# Autodesk Inventor assembly: Assembly1
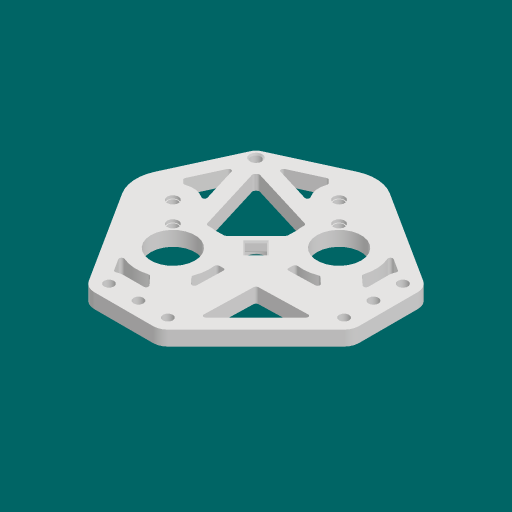
[picture p0: Inventor's stored thumbnail of the model, 512x512]
Saved by Autodesk Inventor 2023.1 (Build 271208000, 208)
## iProperties
Created: 2022-03-15
Part Number: Assembly1
Document SubType Name: Assembly
Designer: zac-h
Author: zac-h
## Documents named in this file (96)
- C:\Users\zac-h\Documents\CAD\guardSwerve1\Assembly1.iam
- C:\Users\zac-h\Documents\CAD\guardSwerve1\Undercarriage.ipt
- C:\Users\zac-h\Documents\CAD\VEX-CAD-Inventor-1.3.0\VEX-CAD-Inventor-1.3.0\Motion\Wheels\Tractions\2.75 Traction, No Insert.ipt
- C:\Users\zac-h\Documents\CAD\guardSwerve1\Assembly1\Design Accelerator\Bevel Gears1.iam
- C:\Users\zac-h\Documents\CAD\VEX-CAD-Inventor-1.3.0\VEX-CAD-Inventor-1.3.0\Motion\Pillow Bearing Block.ipt
- C:\Users\zac-h\Documents\CAD\VEX-CAD-Inventor-1.3.0\VEX-CAD-Inventor-1.3.0\Structure\Hardware\Screw Steel - Star\SScrew Star Smooth .750.ipt
- C:\Users\zac-h\Documents\CAD\VEX-CAD-Inventor-1.3.0\VEX-CAD-Inventor-1.3.0\Structure\Hardware\Screw Steel - Star.ipt
- C:\Users\zac-h\Documents\CAD\guardSwerve1\Assembly1\Design Accelerator\Bevel Gears1_MIR1.iam
- C:\Users\zac-h\Documents\CAD\VEX-CAD-Inventor-1.3.0\VEX-CAD-Inventor-1.3.0\Structure\Hardware\Nut Nylock.ipt
- C:\Users\zac-h\Documents\CAD\VEX-CAD-Inventor-1.3.0\VEX-CAD-Inventor-1.3.0\Electronics\V5 Simple Motor.ipt
- C:\Users\zac-h\Documents\CAD\guardSwerve1\608.ipt
- C:\Users\zac-h\Documents\CAD\guardSwerve1\bearingsleeve.ipt
- C:\Users\zac-h\Documents\CAD\guardSwerve1\lower_plate.ipt
- C:\Users\zac-h\Documents\CAD\guardSwerve1\Assembly1\Design Accelerator\Spur Gears1.iam
- C:\Users\zac-h\Documents\CAD\guardSwerve1\Assembly1\Design Accelerator\Spur Gears2.iam
- C:\Users\zac-h\Documents\CAD\guardSwerve1\Assembly1\Design Accelerator\Spur Gears3.iam
- C:\Users\zac-h\Documents\CAD\guardSwerve1\Assembly1\Design Accelerator\Spur Gears4.iam
- C:\Users\zac-h\Documents\CAD\VEX-CAD-Inventor-1.3.0\VEX-CAD-Inventor-1.3.0\Motion\Shaft LS\Shaft LS 2.5 in.ipt
- C:\Users\zac-h\Documents\CAD\VEX-CAD-Inventor-1.3.0\VEX-CAD-Inventor-1.3.0\Motion\Shaft LS.ipt
- C:\Users\zac-h\Documents\CAD\VEX-CAD-Inventor-1.3.0\VEX-CAD-Inventor-1.3.0\Motion\Shaft Collar with Set Screw.ipt
- C:\Users\zac-h\Documents\CAD\guardSwerve1\vroller.ipt
- C:\Users\zac-h\Documents\CAD\guardSwerve1\upper.ipt
- C:\Users\zac-h\Documents\CAD\guardSwerve1\uppermidblock.ipt
- C:\Users\zac-h\Documents\CAD\guardSwerve1\motorplate.ipt
- C:\Users\zac-h\Documents\CAD\guardSwerve1\Assembly2.iam
- C:\Users\zac-h\Documents\CAD\guardSwerve1\Assembly3.iam
- C:\Users\zac-h\Documents\CAD\guardSwerve1\stls\encoderring.ipt
- C:\Users\zac-h\Documents\CAD\VEX-CAD-Inventor-1.3.0\VEX-CAD-Inventor-1.3.0\Structure\C-Channels\Aluminum 1x2x1\Alu C 1x2x1x26.ipt
- C:\Users\zac-h\Documents\CAD\guardSwerve1\Undercarriage_MIR.ipt
- C:\Users\zac-h\Documents\CAD\VEX-CAD-Inventor-1.3.0\VEX-CAD-Inventor-1.3.0\Motion\Wheels\Tractions\2.75 Traction, No Insert_MIR.ipt
- C:\Users\zac-h\Documents\CAD\guardSwerve1\Assembly1\Design Accelerator\Bevel Gears1_MIR2.iam
- C:\Users\zac-h\Documents\CAD\VEX-CAD-Inventor-1.3.0\VEX-CAD-Inventor-1.3.0\Motion\Pillow Bearing Block_MIR.ipt
- C:\Users\zac-h\Documents\CAD\guardSwerve1\Assembly1\Design Accelerator\Bevel Gears1_MIR1_MIR.iam
- C:\Users\zac-h\Documents\CAD\VEX-CAD-Inventor-1.3.0\VEX-CAD-Inventor-1.3.0\Structure\Hardware\Nut Nylock_MIR.ipt
- C:\Users\zac-h\Documents\CAD\VEX-CAD-Inventor-1.3.0\VEX-CAD-Inventor-1.3.0\Electronics\V5 Simple Motor_MIR.ipt
- C:\Users\zac-h\Documents\CAD\guardSwerve1\608_MIR.ipt
- C:\Users\zac-h\Documents\CAD\guardSwerve1\bearingsleeve_MIR.ipt
- C:\Users\zac-h\Documents\CAD\guardSwerve1\lower_plate_MIR.ipt
- C:\Users\zac-h\Documents\CAD\guardSwerve1\Assembly1\Design Accelerator\Spur Gears1_MIR.iam
- C:\Users\zac-h\Documents\CAD\guardSwerve1\Assembly1\Design Accelerator\Spur Gears2_MIR.iam
- C:\Users\zac-h\Documents\CAD\guardSwerve1\Assembly1\Design Accelerator\Spur Gears3_MIR.iam
- C:\Users\zac-h\Documents\CAD\guardSwerve1\Assembly1\Design Accelerator\Spur Gears4_MIR.iam
- C:\Users\zac-h\Documents\CAD\VEX-CAD-Inventor-1.3.0\VEX-CAD-Inventor-1.3.0\Motion\Shaft Collar with Set Screw_MIR.ipt
- C:\Users\zac-h\Documents\CAD\guardSwerve1\vroller_MIR.ipt
- C:\Users\zac-h\Documents\CAD\guardSwerve1\upper_MIR.ipt
- C:\Users\zac-h\Documents\CAD\guardSwerve1\uppermidblock_MIR.ipt
- C:\Users\zac-h\Documents\CAD\guardSwerve1\motorplate_MIR.ipt
- C:\Users\zac-h\Documents\CAD\guardSwerve1\Assembly2_MIR.iam
- C:\Users\zac-h\Documents\CAD\guardSwerve1\Assembly3_MIR.iam
- C:\Users\zac-h\Documents\CAD\guardSwerve1\stls\encoderring_MIR.ipt
- C:\Users\zac-h\Documents\CAD\guardSwerve1\Undercarriage_MIR1.ipt
- C:\Users\zac-h\Documents\CAD\VEX-CAD-Inventor-1.3.0\VEX-CAD-Inventor-1.3.0\Motion\Wheels\Tractions\2.75 Traction, No Insert_MIR1.ipt
- C:\Users\zac-h\Documents\CAD\guardSwerve1\Assembly1\Design Accelerator\Bevel Gears1_MIR3.iam
- C:\Users\zac-h\Documents\CAD\VEX-CAD-Inventor-1.3.0\VEX-CAD-Inventor-1.3.0\Motion\Pillow Bearing Block_MIR1.ipt
- C:\Users\zac-h\Documents\CAD\guardSwerve1\Assembly1\Design Accelerator\Bevel Gears1_MIR1_MIR1.iam
- C:\Users\zac-h\Documents\CAD\VEX-CAD-Inventor-1.3.0\VEX-CAD-Inventor-1.3.0\Structure\Hardware\Nut Nylock_MIR1.ipt
- C:\Users\zac-h\Documents\CAD\VEX-CAD-Inventor-1.3.0\VEX-CAD-Inventor-1.3.0\Electronics\V5 Simple Motor_MIR1.ipt
- C:\Users\zac-h\Documents\CAD\guardSwerve1\608_MIR1.ipt
- C:\Users\zac-h\Documents\CAD\guardSwerve1\bearingsleeve_MIR1.ipt
- C:\Users\zac-h\Documents\CAD\guardSwerve1\lower_plate_MIR1.ipt
- C:\Users\zac-h\Documents\CAD\guardSwerve1\Assembly1\Design Accelerator\Spur Gears1_MIR1.iam
- C:\Users\zac-h\Documents\CAD\guardSwerve1\Assembly1\Design Accelerator\Spur Gears2_MIR1.iam
- C:\Users\zac-h\Documents\CAD\guardSwerve1\Assembly1\Design Accelerator\Spur Gears3_MIR1.iam
- C:\Users\zac-h\Documents\CAD\guardSwerve1\Assembly1\Design Accelerator\Spur Gears4_MIR1.iam
- C:\Users\zac-h\Documents\CAD\VEX-CAD-Inventor-1.3.0\VEX-CAD-Inventor-1.3.0\Motion\Shaft Collar with Set Screw_MIR1.ipt
- C:\Users\zac-h\Documents\CAD\guardSwerve1\vroller_MIR1.ipt
- C:\Users\zac-h\Documents\CAD\guardSwerve1\upper_MIR1.ipt
- C:\Users\zac-h\Documents\CAD\guardSwerve1\uppermidblock_MIR1.ipt
- C:\Users\zac-h\Documents\CAD\guardSwerve1\motorplate_MIR1.ipt
- C:\Users\zac-h\Documents\CAD\guardSwerve1\Assembly2_MIR1.iam
- C:\Users\zac-h\Documents\CAD\guardSwerve1\Assembly3_MIR1.iam
- C:\Users\zac-h\Documents\CAD\guardSwerve1\stls\encoderring_MIR1.ipt
- C:\Users\zac-h\Documents\CAD\VEX-CAD-Inventor-1.3.0\VEX-CAD-Inventor-1.3.0\Structure\C-Channels\Aluminum 1x2x1\Alu C 1x2x1x26_MIR.ipt
- C:\Users\zac-h\Documents\CAD\guardSwerve1\Undercarriage_MIR_MIR.ipt
- C:\Users\zac-h\Documents\CAD\VEX-CAD-Inventor-1.3.0\VEX-CAD-Inventor-1.3.0\Motion\Wheels\Tractions\2.75 Traction, No Insert_MIR_MIR.ipt
- C:\Users\zac-h\Documents\CAD\guardSwerve1\Assembly1\Design Accelerator\Bevel Gears1_MIR2_MIR.iam
- C:\Users\zac-h\Documents\CAD\VEX-CAD-Inventor-1.3.0\VEX-CAD-Inventor-1.3.0\Motion\Pillow Bearing Block_MIR_MIR.ipt
- C:\Users\zac-h\Documents\CAD\guardSwerve1\Assembly1\Design Accelerator\Bevel Gears1_MIR1_MIR_MIR.iam
- C:\Users\zac-h\Documents\CAD\VEX-CAD-Inventor-1.3.0\VEX-CAD-Inventor-1.3.0\Structure\Hardware\Nut Nylock_MIR_MIR.ipt
- C:\Users\zac-h\Documents\CAD\VEX-CAD-Inventor-1.3.0\VEX-CAD-Inventor-1.3.0\Electronics\V5 Simple Motor_MIR_MIR.ipt
- C:\Users\zac-h\Documents\CAD\guardSwerve1\608_MIR_MIR.ipt
- C:\Users\zac-h\Documents\CAD\guardSwerve1\bearingsleeve_MIR_MIR.ipt
- C:\Users\zac-h\Documents\CAD\guardSwerve1\lower_plate_MIR_MIR.ipt
- C:\Users\zac-h\Documents\CAD\guardSwerve1\Assembly1\Design Accelerator\Spur Gears1_MIR_MIR.iam
- C:\Users\zac-h\Documents\CAD\guardSwerve1\Assembly1\Design Accelerator\Spur Gears2_MIR_MIR.iam
- C:\Users\zac-h\Documents\CAD\guardSwerve1\Assembly1\Design Accelerator\Spur Gears3_MIR_MIR.iam
- C:\Users\zac-h\Documents\CAD\guardSwerve1\Assembly1\Design Accelerator\Spur Gears4_MIR_MIR.iam
- C:\Users\zac-h\Documents\CAD\VEX-CAD-Inventor-1.3.0\VEX-CAD-Inventor-1.3.0\Motion\Shaft Collar with Set Screw_MIR_MIR.ipt
- C:\Users\zac-h\Documents\CAD\guardSwerve1\upper_MIR_MIR.ipt
- C:\Users\zac-h\Documents\CAD\guardSwerve1\uppermidblock_MIR_MIR.ipt
- C:\Users\zac-h\Documents\CAD\guardSwerve1\motorplate_MIR_MIR.ipt
- C:\Users\zac-h\Documents\CAD\guardSwerve1\Assembly2_MIR_MIR.iam
- C:\Users\zac-h\Documents\CAD\guardSwerve1\Assembly3_MIR_MIR.iam
- C:\Users\zac-h\Documents\CAD\guardSwerve1\stls\encoderring_MIR_MIR.ipt
- C:\Users\zac-h\Documents\CAD\guardSwerve1\vroller_MIR_MIR.ipt
- C:\Users\zac-h\Documents\CAD\VEX-CAD-Inventor-1.3.0\VEX-CAD-Inventor-1.3.0\Structure\C-Channels\Aluminum 1x2x1\Alu C 1x2x1x26_MIR_MIR.ipt
## Components (189 placed, 90 different names)
1. Undercarriage:1 — Mate:1, Insert:1, Insert:2, Insert:3, Insert:4, Insert:5, Insert:6, Insert:7, Insert:8, Flush:1, Insert:13, Insert:14, Flush:2, Flush:3, Insert:19, Mate:42, Mate:46, Mate:50, Mate:53, Flush:11
2. 2.75 Traction, No Insert:1 — Rigid:1, Mate:1, Mate:4
3. Bevel Gears:1 [sub-assembly] — Rigid:1, Mate:2, Mate:3, Angle:1, Angle:2
4. Pillow Bearing Block:1 — Insert:5, Insert:6, Insert:9, Insert:10, Insert:28
5. Pillow Bearing Block:2 — Insert:1, Insert:2, Mate:2, Insert:11, Insert:12, Insert:29
6. SScrew Star Smooth .750:1 — Insert:3
7. SScrew Star Smooth .750:2 — Insert:4
8. SScrew Star Smooth .750:3 — Insert:7
9. SScrew Star Smooth .750:4 — Insert:8
10. Bevel Gears1_MIR1:1 [sub-assembly] — Mate:3, Angle:1, Mate:4
11. Nut Nylock:1 — Insert:9
12. Nut Nylock:2 — Insert:11
13. Nut Nylock:3 — Insert:10
14. Nut Nylock:4 — Insert:12
15. V5 Simple Motor:1 — Insert:39, Insert:40
16. V5 Simple Motor:2 — Insert:37, Insert:38
17. 608:1 — Flush:1, Insert:14, Insert:21
18. 608:2 — Insert:13, Insert:15
19. bearingsleeve:1 — Insert:15, Mate:44, Mate:47
20. lower_plate:1 — Flush:2, Flush:3, Insert:32, Insert:33, Insert:34, Flush:6, Flush:7, Insert:41, Insert:42, Insert:43
21. Spur Gears:1 [sub-assembly] — Mate:44, Mate:45, Mate:46, Mate:47, Mate:49, Mate:51
22. 608:3 — Insert:19, Insert:20
23. bearingsleeve:2 — Insert:20, Mate:45
24. bearingsleeve:3 — Insert:21, Mate:48
25. Spur Gears:2 [sub-assembly] — Mate:48, Mate:49, Mate:50, Mate:51, Insert:31, Mate:54
26. Spur Gears:3 [sub-assembly] — Insert:26, Mate:53, Mate:54
27. 608:4 — Insert:24, Insert:31
28. 608:5 — Insert:25, Insert:26
29. bearingsleeve:4 — Insert:24
30. bearingsleeve:5 — Insert:25, Mate:43
31. Spur Gears:4 [sub-assembly] — Mate:42, Mate:43, Mate:52
32. Shaft LS 2.5 in:1 — Insert:30
33. Shaft Collar with Set Screw:1 — Insert:29, Insert:30
34. Shaft Collar with Set Screw:2 — Insert:28
35. 608:6 — Insert:32
36. 608:7 — Insert:33
37. 608:8 — Insert:34, Flush:4, Flush:5, Insert:36
38. midblock — Flush:6, Flush:7, Flush:8, Flush:9
39. uppermidblock:1 — Flush:8, Flush:9, Flush:10, Angle:3
40. motorplate:1 — Flush:10, Insert:37, Insert:38, Insert:39, Insert:40
41. Assembly2:1 [sub-assembly]
42. Assembly3:1 [sub-assembly]
43. encoderring:1 — Flush:11
44. Alu C 1x2x1x26:1 — Insert:41
45. Alu C 1x2x1x26:2 — Insert:42, Insert:43
46. Undercarriage_MIR:1 — Mate:55, Insert:44, Insert:45, Insert:46, Insert:47, Insert:48, Insert:49, Insert:50, Insert:51, Insert:56, Mate:59, Insert:57, Mate:60, Mate:61, Mate:63, Insert:59, Mate:67, Mate:71, Mate:73, Mate:82
47. 2.75 Traction, No Insert_MIR:1 — Mate:55, Mate:57, Rigid:2
48. Bevel Gears1_MIR2:1 [sub-assembly] — Mate:56, Mate:58, Angle:4, Angle:5, Rigid:2
49. Pillow Bearing Block_MIR:1 — Insert:44, Insert:45, Insert:52, Insert:54, Insert:68
50. Pillow Bearing Block_MIR:2 — Mate:56, Insert:46, Insert:47, Insert:53, Insert:55, Insert:67
51. SScrew Star Smooth .750:5 — Insert:48
52. SScrew Star Smooth .750:6 — Insert:49
53. SScrew Star Smooth .750:7 — Insert:50
54. SScrew Star Smooth .750:8 — Insert:51
55. Bevel Gears1_MIR1_MIR:1 [sub-assembly] — Mate:57, Mate:58, Angle:4
56. Nut Nylock_MIR:1 — Insert:52
57. Nut Nylock_MIR:2 — Insert:53
58. Nut Nylock_MIR:3 — Insert:54
59. Nut Nylock_MIR:4 — Insert:55
60. V5 Simple Motor_MIR:1 — Insert:73, Insert:74
61. V5 Simple Motor_MIR:2 — Insert:75, Insert:76
62. 608_MIR:1 — Insert:56, Mate:59, Insert:61
63. 608_MIR:2 — Insert:57, Insert:58
64. bearingsleeve_MIR:1 — Insert:58, Mate:62, Mate:64
65. lower_plate_MIR:1 — Mate:60, Mate:61, Insert:69, Insert:70, Insert:71, Mate:76, Mate:77
66. Spur Gears1_MIR:1 [sub-assembly] — Mate:62, Mate:63, Mate:64, Mate:65, Mate:66, Mate:68
67. 608_MIR:3 — Insert:59, Insert:60
68. bearingsleeve_MIR:2 — Mate:65, Insert:60
69. bearingsleeve_MIR:3 — Insert:61, Mate:69
70. Spur Gears2_MIR:1 [sub-assembly] — Mate:66, Mate:67, Mate:68, Mate:69, Mate:70, Insert:62
71. Spur Gears3_MIR:1 [sub-assembly] — Mate:70, Mate:71, Insert:63
72. 608_MIR:4 — Insert:62, Insert:64
73. 608_MIR:5 — Insert:63, Insert:65
74. bearingsleeve_MIR:4 — Insert:64
75. bearingsleeve_MIR:5 — Insert:65, Mate:72
76. Spur Gears4_MIR:1 [sub-assembly] — Mate:72, Mate:73, Mate:81
77. Shaft LS 2.5 in:2 — Insert:66
78. Shaft Collar with Set Screw_MIR:1 — Insert:66, Insert:67
79. Shaft Collar with Set Screw_MIR:2 — Insert:68
80. 608_MIR:6 — Insert:69
81. 608_MIR:7 — Insert:70
82. 608_MIR:8 — Insert:71, Insert:72, Mate:74, Mate:75
83. upper_MIR:1 — Mate:76, Mate:77, Mate:78, Mate:79
84. uppermidblock_MIR:1 — Mate:78, Mate:79, Mate:80, Angle:6
85. motorplate_MIR:1 — Insert:73, Insert:74, Insert:75, Insert:76, Mate:80
86. Assembly2_MIR:1 [sub-assembly]
87. Assembly3_MIR:1 [sub-assembly]
88. encoderring_MIR:1 — Mate:82
89. Undercarriage_MIR1:1 — Mate:83, Insert:77, Insert:78, Insert:79, Insert:80, Insert:81, Insert:82, Insert:83, Insert:84, Insert:89, Mate:87, Insert:90, Mate:88, Mate:89, Mate:91, Insert:92, Mate:95, Mate:99, Mate:101, Mate:110
90. 2.75 Traction, No Insert_MIR1:1 — Mate:83, Mate:85, Rigid:3
91. Bevel Gears1_MIR3:1 [sub-assembly] — Mate:84, Mate:86, Angle:7, Angle:8, Rigid:3
92. Pillow Bearing Block_MIR1:1 — Insert:77, Insert:78, Insert:85, Insert:87, Insert:101
93. Pillow Bearing Block_MIR1:2 — Mate:84, Insert:79, Insert:80, Insert:86, Insert:88, Insert:100
94. SScrew Star Smooth .750:9 — Insert:81
95. SScrew Star Smooth .750:10 — Insert:82
96. SScrew Star Smooth .750:11 — Insert:83
97. SScrew Star Smooth .750:12 — Insert:84
98. Bevel Gears1_MIR1_MIR1:1 [sub-assembly] — Mate:85, Mate:86, Angle:7
99. Nut Nylock_MIR1:1 — Insert:85
100. Nut Nylock_MIR1:2 — Insert:86
101. Nut Nylock_MIR1:3 — Insert:87
102. Nut Nylock_MIR1:4 — Insert:88
103. V5 Simple Motor_MIR1:1 — Insert:106, Insert:107
104. V5 Simple Motor_MIR1:2 — Insert:108, Insert:109
105. 608_MIR1:1 — Insert:89, Mate:87, Insert:94
106. 608_MIR1:2 — Insert:90, Insert:91
107. bearingsleeve_MIR1:1 — Insert:91, Mate:90, Mate:92
108. lower_plate_MIR1:1 — Mate:88, Mate:89, Insert:102, Insert:103, Insert:104, Mate:104, Mate:105, Insert:110, Insert:111, Insert:112
109. Spur Gears1_MIR1:1 [sub-assembly] — Mate:90, Mate:91, Mate:92, Mate:93, Mate:94, Mate:96
110. 608_MIR1:3 — Insert:92, Insert:93
111. bearingsleeve_MIR1:2 — Mate:93, Insert:93
112. bearingsleeve_MIR1:3 — Insert:94, Mate:97
113. Spur Gears2_MIR1:1 [sub-assembly] — Mate:94, Mate:95, Mate:96, Mate:97, Mate:98, Insert:95
114. Spur Gears3_MIR1:1 [sub-assembly] — Mate:98, Mate:99, Insert:96
115. 608_MIR1:4 — Insert:95, Insert:97
116. 608_MIR1:5 — Insert:96, Insert:98
117. bearingsleeve_MIR1:4 — Insert:97
118. bearingsleeve_MIR1:5 — Insert:98, Mate:100
119. Spur Gears4_MIR1:1 [sub-assembly] — Mate:100, Mate:101, Mate:109
120. Shaft LS 2.5 in:3 — Insert:99
121. Shaft Collar with Set Screw_MIR1:1 — Insert:99, Insert:100
122. Shaft Collar with Set Screw_MIR1:2 — Insert:101
123. 608_MIR1:6 — Insert:102
124. 608_MIR1:7 — Insert:103
125. 608_MIR1:8 — Insert:104, Insert:105, Mate:102, Mate:103
126. upper_MIR1:1 — Mate:104, Mate:105, Mate:106, Mate:107
127. uppermidblock_MIR1:1 — Mate:106, Mate:107, Mate:108, Angle:9
128. motorplate_MIR1:1 — Insert:106, Insert:107, Insert:108, Insert:109, Mate:108
129. Assembly2_MIR1:1 [sub-assembly]
130. Assembly3_MIR1:1 [sub-assembly]
131. encoderring_MIR1:1 — Mate:110
132. Alu C 1x2x1x26_MIR:1 — Insert:110
133. Alu C 1x2x1x26_MIR:2 — Insert:111, Insert:112
134. Undercarriage_MIR_MIR:1 — Mate:111, Insert:113, Insert:114, Insert:115, Insert:116, Insert:117, Insert:118, Insert:119, Insert:120, Flush:12, Insert:125, Insert:126, Flush:13, Flush:14, Mate:116, Insert:128, Mate:121, Mate:123, Mate:125, Flush:22
135. 2.75 Traction, No Insert_MIR_MIR:1 — Mate:111, Mate:114, Rigid:4
136. Bevel Gears1_MIR2_MIR:1 [sub-assembly] — Mate:112, Mate:113, Angle:10, Angle:11, Rigid:4
137. Pillow Bearing Block_MIR_MIR:1 — Insert:113, Insert:114, Insert:121, Insert:123, Insert:137
138. Pillow Bearing Block_MIR_MIR:2 — Insert:115, Insert:116, Mate:112, Insert:122, Insert:124, Insert:135
139. SScrew Star Smooth .750:13 — Insert:117
140. SScrew Star Smooth .750:14 — Insert:118
141. SScrew Star Smooth .750:15 — Insert:119
142. SScrew Star Smooth .750:16 — Insert:120
143. Bevel Gears1_MIR1_MIR_MIR:1 [sub-assembly] — Mate:113, Mate:114, Angle:10
144. Nut Nylock_MIR_MIR:1 — Insert:121
145. Nut Nylock_MIR_MIR:2 — Insert:122
146. Nut Nylock_MIR_MIR:3 — Insert:123
147. Nut Nylock_MIR_MIR:4 — Insert:124
148. V5 Simple Motor_MIR_MIR:1 — Insert:144, Insert:145
149. V5 Simple Motor_MIR_MIR:2 — Insert:142, Insert:143
150. 608_MIR_MIR:1 — Flush:12, Insert:125, Insert:130
151. 608_MIR_MIR:2 — Insert:126, Insert:127
152. bearingsleeve_MIR_MIR:1 — Insert:127, Mate:115, Mate:117
153. lower_plate_MIR_MIR:1 — Flush:13, Flush:14, Insert:138, Insert:139, Insert:140, Flush:17, Flush:18
154. Spur Gears1_MIR_MIR:1 [sub-assembly] — Mate:115, Mate:116, Mate:117, Mate:118, Mate:120, Mate:122
155. 608_MIR_MIR:3 — Insert:128, Insert:129
156. bearingsleeve_MIR_MIR:2 — Insert:129, Mate:118
157. bearingsleeve_MIR_MIR:3 — Insert:130, Mate:119
158. Spur Gears2_MIR_MIR:1 [sub-assembly] — Mate:119, Mate:120, Mate:121, Mate:122, Mate:124, Insert:131
159. Spur Gears3_MIR_MIR:1 [sub-assembly] — Mate:123, Mate:124, Insert:132
160. 608_MIR_MIR:4 — Insert:131, Insert:133
161. 608_MIR_MIR:5 — Insert:132, Insert:134
162. bearingsleeve_MIR_MIR:4 — Insert:133
163. bearingsleeve_MIR_MIR:5 — Insert:134, Mate:126
164. Spur Gears4_MIR_MIR:1 [sub-assembly] — Mate:125, Mate:126, Mate:127
165. Shaft LS 2.5 in:4 — Insert:136
166. Shaft Collar with Set Screw_MIR_MIR:1 — Insert:135, Insert:136
167. Shaft Collar with Set Screw_MIR_MIR:2 — Insert:137
168. 608_MIR_MIR:6 — Insert:138
169. 608_MIR_MIR:7 — Insert:139
170. 608_MIR_MIR:8 — Insert:140, Flush:15, Flush:16, Insert:141
171. upper_MIR_MIR:1 — Flush:17, Flush:18, Flush:19, Flush:20
172. uppermidblock_MIR_MIR:1 — Flush:19, Flush:20, Flush:21, Angle:12
173. motorplate_MIR_MIR:1 — Flush:21, Insert:142, Insert:143, Insert:144, Insert:145
174. Assembly2_MIR_MIR:1 [sub-assembly]
175. Assembly3_MIR_MIR:1 [sub-assembly]
176. encoderring_MIR_MIR:1 — Flush:22
177. Alu C 1x2x1x26_MIR_MIR:1
178. vroller:1 — Flush:4, Flush:5, Insert:36
179. vroller:2
180. vroller:3
181. vroller_MIR:1 — Insert:72, Mate:74, Mate:75
182. vroller_MIR:2
183. vroller_MIR:3
184. vroller_MIR1:1 — Insert:105, Mate:102, Mate:103
185. vroller_MIR1:2
186. vroller_MIR1:3
187. vroller_MIR_MIR:1 — Flush:15, Flush:16, Insert:141
188. vroller_MIR_MIR:2
189. vroller_MIR_MIR:3
## Component patterns: (3 elements, first: vroller:1), (3 elements, first: vroller_MIR:1), (3 elements, first: vroller_MIR1:1), (3 elements, first: vroller_MIR_MIR:1)
## Relationships (266: Insert 138, Mate 90, Flush 22, Angle 12, WeldJoint 4)
- Rigid:1 [WeldJoint]: 2.75 Traction, No Insert:1 ↔ Bevel Gears:1
- Mate:1: Undercarriage:1 ↔ 2.75 Traction, No Insert:1
- Insert:1: Undercarriage:1 ↔ Pillow Bearing Block:2
- Insert:2: Undercarriage:1 ↔ Pillow Bearing Block:2
- Mate:2: Bevel Gears:1 ↔ Pillow Bearing Block:2
- Insert:3: Undercarriage:1 ↔ SScrew Star Smooth .750:1
- Insert:4: Undercarriage:1 ↔ SScrew Star Smooth .750:2
- Mate:3: Bevel Gears:1 ↔ Bevel Gears1_MIR1:1
- Angle:1 (0 deg): Bevel Gears:1 ↔ Bevel Gears1_MIR1:1
- Mate:4: 2.75 Traction, No Insert:1 ↔ Bevel Gears1_MIR1:1
- Angle:2 (180 deg): Bevel Gears:1
- Insert:5: Undercarriage:1 ↔ Pillow Bearing Block:1
- Insert:6: Undercarriage:1 ↔ Pillow Bearing Block:1
- Insert:7: Undercarriage:1 ↔ SScrew Star Smooth .750:3
- Insert:8: Undercarriage:1 ↔ SScrew Star Smooth .750:4
- Insert:9: Pillow Bearing Block:1 ↔ Nut Nylock:1
- Insert:10: Pillow Bearing Block:1 ↔ Nut Nylock:3
- Insert:11: Pillow Bearing Block:2 ↔ Nut Nylock:2
- Insert:12: Pillow Bearing Block:2 ↔ Nut Nylock:4
- Flush:1: Undercarriage:1 ↔ 608:1
- Insert:13: Undercarriage:1 ↔ 608:2
- Insert:14: Undercarriage:1 ↔ 608:1
- Insert:15: 608:2 ↔ bearingsleeve:1
- Flush:2: Undercarriage:1 ↔ lower_plate:1
- Flush:3 (3 mm): Undercarriage:1 ↔ lower_plate:1
- Insert:19: Undercarriage:1 ↔ 608:3
- Insert:20: 608:3 ↔ bearingsleeve:2
- Insert:21: 608:1 ↔ bearingsleeve:3
- Insert:24: 608:4 ↔ bearingsleeve:4
- Insert:25: 608:5 ↔ bearingsleeve:5
- Mate:42: Undercarriage:1 ↔ Spur Gears:4
- Mate:43: bearingsleeve:5 ↔ Spur Gears:4
- Insert:26: Spur Gears:3 ↔ 608:5
- Insert:28: Pillow Bearing Block:1 ↔ Shaft Collar with Set Screw:2
- Insert:29: Pillow Bearing Block:2 ↔ Shaft Collar with Set Screw:1
- Insert:30: Shaft LS 2.5 in:1 ↔ Shaft Collar with Set Screw:1
- Mate:44: bearingsleeve:1 ↔ Spur Gears:1
- Mate:45 (1.5875 mm): Spur Gears:1 ↔ bearingsleeve:2
- Mate:46: Undercarriage:1 ↔ Spur Gears:1
- Mate:47 (1.5875 mm): bearingsleeve:1 ↔ Spur Gears:1
- Mate:48: bearingsleeve:3 ↔ Spur Gears:2
- Mate:49 (1.5875 mm): Spur Gears:1 ↔ Spur Gears:2
- Mate:50: Undercarriage:1 ↔ Spur Gears:2
- Mate:51 (1.5875 mm): Spur Gears:1 ↔ Spur Gears:2
- Insert:31: Spur Gears:2 ↔ 608:4
- Insert:32: lower_plate:1 ↔ 608:6
- Insert:33: lower_plate:1 ↔ 608:7
- Insert:34: lower_plate:1 ↔ 608:8
- Flush:4: 608:8 ↔ vroller:1
- Flush:5: 608:8 ↔ vroller:1
- Flush:6: lower_plate:1 ↔ midblock
- Flush:7: lower_plate:1 ↔ midblock
- Insert:36: 608:8 ↔ vroller:1
- Flush:8: midblock ↔ uppermidblock:1
- Flush:9: midblock ↔ uppermidblock:1
- Flush:10: uppermidblock:1 ↔ motorplate:1
- Insert:37: V5 Simple Motor:2 ↔ motorplate:1
- Insert:38: V5 Simple Motor:2 ↔ motorplate:1
- Insert:39: V5 Simple Motor:1 ↔ motorplate:1
- Insert:40: V5 Simple Motor:1 ↔ motorplate:1
- Mate:52: Spur Gears:4
- Angle:3 (90 deg): uppermidblock:1
- Mate:53: Undercarriage:1 ↔ Spur Gears:3
- Mate:54: Spur Gears:2 ↔ Spur Gears:3
- Flush:11: Undercarriage:1 ↔ encoderring:1
- Insert:41: lower_plate:1 ↔ Alu C 1x2x1x26:1
- Insert:42: lower_plate:1 ↔ Alu C 1x2x1x26:2
- Insert:43: lower_plate:1 ↔ Alu C 1x2x1x26:2
- Mate:55: Undercarriage_MIR:1 ↔ 2.75 Traction, No Insert_MIR:1
- Insert:44: Undercarriage_MIR:1 ↔ Pillow Bearing Block_MIR:1
- Insert:45: Undercarriage_MIR:1 ↔ Pillow Bearing Block_MIR:1
- Mate:56: Bevel Gears1_MIR2:1 ↔ Pillow Bearing Block_MIR:2
- Insert:46: Undercarriage_MIR:1 ↔ Pillow Bearing Block_MIR:2
- Insert:47: Undercarriage_MIR:1 ↔ Pillow Bearing Block_MIR:2
- Insert:48: Undercarriage_MIR:1 ↔ SScrew Star Smooth .750:5
- Insert:49: Undercarriage_MIR:1 ↔ SScrew Star Smooth .750:6
- Insert:50: Undercarriage_MIR:1 ↔ SScrew Star Smooth .750:7
- Insert:51: Undercarriage_MIR:1 ↔ SScrew Star Smooth .750:8
- Mate:57: 2.75 Traction, No Insert_MIR:1 ↔ Bevel Gears1_MIR1_MIR:1
- Mate:58: Bevel Gears1_MIR2:1 ↔ Bevel Gears1_MIR1_MIR:1
- Angle:4 (0 deg): Bevel Gears1_MIR2:1 ↔ Bevel Gears1_MIR1_MIR:1
- Angle:5 (180 deg): Bevel Gears1_MIR2:1
- Insert:52: Pillow Bearing Block_MIR:1 ↔ Nut Nylock_MIR:1
- Insert:53: Pillow Bearing Block_MIR:2 ↔ Nut Nylock_MIR:2
- Insert:54: Pillow Bearing Block_MIR:1 ↔ Nut Nylock_MIR:3
- Insert:55: Pillow Bearing Block_MIR:2 ↔ Nut Nylock_MIR:4
- Insert:56: Undercarriage_MIR:1 ↔ 608_MIR:1
- Mate:59: Undercarriage_MIR:1 ↔ 608_MIR:1
- Insert:57: Undercarriage_MIR:1 ↔ 608_MIR:2
- Insert:58: 608_MIR:2 ↔ bearingsleeve_MIR:1
- Mate:60 (3 mm): Undercarriage_MIR:1 ↔ lower_plate_MIR:1
- Mate:61: Undercarriage_MIR:1 ↔ lower_plate_MIR:1
- Mate:62 (1.5875 mm): bearingsleeve_MIR:1 ↔ Spur Gears1_MIR:1
- Mate:63: Undercarriage_MIR:1 ↔ Spur Gears1_MIR:1
- Mate:64: bearingsleeve_MIR:1 ↔ Spur Gears1_MIR:1
- Insert:59: Undercarriage_MIR:1 ↔ 608_MIR:3
- Mate:65 (1.5875 mm): Spur Gears1_MIR:1 ↔ bearingsleeve_MIR:2
- Insert:60: 608_MIR:3 ↔ bearingsleeve_MIR:2
- Insert:61: 608_MIR:1 ↔ bearingsleeve_MIR:3
- Mate:66 (1.5875 mm): Spur Gears1_MIR:1 ↔ Spur Gears2_MIR:1
- Mate:67: Undercarriage_MIR:1 ↔ Spur Gears2_MIR:1
- Mate:68 (1.5875 mm): Spur Gears1_MIR:1 ↔ Spur Gears2_MIR:1
- Mate:69: bearingsleeve_MIR:3 ↔ Spur Gears2_MIR:1
- Mate:70: Spur Gears2_MIR:1 ↔ Spur Gears3_MIR:1
- Mate:71: Undercarriage_MIR:1 ↔ Spur Gears3_MIR:1
- Insert:62: Spur Gears2_MIR:1 ↔ 608_MIR:4
- Insert:63: Spur Gears3_MIR:1 ↔ 608_MIR:5
- Insert:64: 608_MIR:4 ↔ bearingsleeve_MIR:4
- Insert:65: 608_MIR:5 ↔ bearingsleeve_MIR:5
- Mate:72: bearingsleeve_MIR:5 ↔ Spur Gears4_MIR:1
- Mate:73: Undercarriage_MIR:1 ↔ Spur Gears4_MIR:1
- Insert:66: Shaft LS 2.5 in:2 ↔ Shaft Collar with Set Screw_MIR:1
- Insert:67: Pillow Bearing Block_MIR:2 ↔ Shaft Collar with Set Screw_MIR:1
- Insert:68: Pillow Bearing Block_MIR:1 ↔ Shaft Collar with Set Screw_MIR:2
- Insert:69: lower_plate_MIR:1 ↔ 608_MIR:6
- Insert:70: lower_plate_MIR:1 ↔ 608_MIR:7
- Insert:71: lower_plate_MIR:1 ↔ 608_MIR:8
- Insert:72: 608_MIR:8 ↔ vroller_MIR:1
- Mate:74: 608_MIR:8 ↔ vroller_MIR:1
- Mate:75: 608_MIR:8 ↔ vroller_MIR:1
- Mate:76: lower_plate_MIR:1 ↔ upper_MIR:1
- Mate:77: lower_plate_MIR:1 ↔ upper_MIR:1
- Mate:78: upper_MIR:1 ↔ uppermidblock_MIR:1
- Mate:79: upper_MIR:1 ↔ uppermidblock_MIR:1
- Insert:73: V5 Simple Motor_MIR:1 ↔ motorplate_MIR:1
- Insert:74: V5 Simple Motor_MIR:1 ↔ motorplate_MIR:1
- Insert:75: V5 Simple Motor_MIR:2 ↔ motorplate_MIR:1
- Insert:76: V5 Simple Motor_MIR:2 ↔ motorplate_MIR:1
- Mate:80: uppermidblock_MIR:1 ↔ motorplate_MIR:1
- Mate:81: Spur Gears4_MIR:1
- Angle:6 (-90 deg): uppermidblock_MIR:1
- Mate:82: Undercarriage_MIR:1 ↔ encoderring_MIR:1
- Rigid:2 [WeldJoint]: 2.75 Traction, No Insert_MIR:1 ↔ Bevel Gears1_MIR2:1
- Mate:83: Undercarriage_MIR1:1 ↔ 2.75 Traction, No Insert_MIR1:1
- Insert:77: Undercarriage_MIR1:1 ↔ Pillow Bearing Block_MIR1:1
- Insert:78: Undercarriage_MIR1:1 ↔ Pillow Bearing Block_MIR1:1
- Mate:84: Bevel Gears1_MIR3:1 ↔ Pillow Bearing Block_MIR1:2
- Insert:79: Undercarriage_MIR1:1 ↔ Pillow Bearing Block_MIR1:2
- Insert:80: Undercarriage_MIR1:1 ↔ Pillow Bearing Block_MIR1:2
- Insert:81: Undercarriage_MIR1:1 ↔ SScrew Star Smooth .750:9
- Insert:82: Undercarriage_MIR1:1 ↔ SScrew Star Smooth .750:10
- Insert:83: Undercarriage_MIR1:1 ↔ SScrew Star Smooth .750:11
- Insert:84: Undercarriage_MIR1:1 ↔ SScrew Star Smooth .750:12
- Mate:85: 2.75 Traction, No Insert_MIR1:1 ↔ Bevel Gears1_MIR1_MIR1:1
- Mate:86: Bevel Gears1_MIR3:1 ↔ Bevel Gears1_MIR1_MIR1:1
- Angle:7 (0 deg): Bevel Gears1_MIR3:1 ↔ Bevel Gears1_MIR1_MIR1:1
- Angle:8 (180 deg): Bevel Gears1_MIR3:1
- Insert:85: Pillow Bearing Block_MIR1:1 ↔ Nut Nylock_MIR1:1
- Insert:86: Pillow Bearing Block_MIR1:2 ↔ Nut Nylock_MIR1:2
- Insert:87: Pillow Bearing Block_MIR1:1 ↔ Nut Nylock_MIR1:3
- Insert:88: Pillow Bearing Block_MIR1:2 ↔ Nut Nylock_MIR1:4
- Insert:89: Undercarriage_MIR1:1 ↔ 608_MIR1:1
- Mate:87: Undercarriage_MIR1:1 ↔ 608_MIR1:1
- Insert:90: Undercarriage_MIR1:1 ↔ 608_MIR1:2
- Insert:91: 608_MIR1:2 ↔ bearingsleeve_MIR1:1
- Mate:88 (3 mm): Undercarriage_MIR1:1 ↔ lower_plate_MIR1:1
- Mate:89: Undercarriage_MIR1:1 ↔ lower_plate_MIR1:1
- Mate:90 (1.5875 mm): bearingsleeve_MIR1:1 ↔ Spur Gears1_MIR1:1
- Mate:91: Undercarriage_MIR1:1 ↔ Spur Gears1_MIR1:1
- Mate:92: bearingsleeve_MIR1:1 ↔ Spur Gears1_MIR1:1
- Insert:92: Undercarriage_MIR1:1 ↔ 608_MIR1:3
- Mate:93 (1.5875 mm): Spur Gears1_MIR1:1 ↔ bearingsleeve_MIR1:2
- Insert:93: 608_MIR1:3 ↔ bearingsleeve_MIR1:2
- Insert:94: 608_MIR1:1 ↔ bearingsleeve_MIR1:3
- Mate:94 (1.5875 mm): Spur Gears1_MIR1:1 ↔ Spur Gears2_MIR1:1
- Mate:95: Undercarriage_MIR1:1 ↔ Spur Gears2_MIR1:1
- Mate:96 (1.5875 mm): Spur Gears1_MIR1:1 ↔ Spur Gears2_MIR1:1
- Mate:97: bearingsleeve_MIR1:3 ↔ Spur Gears2_MIR1:1
- Mate:98: Spur Gears2_MIR1:1 ↔ Spur Gears3_MIR1:1
- Mate:99: Undercarriage_MIR1:1 ↔ Spur Gears3_MIR1:1
- Insert:95: Spur Gears2_MIR1:1 ↔ 608_MIR1:4
- Insert:96: Spur Gears3_MIR1:1 ↔ 608_MIR1:5
- Insert:97: 608_MIR1:4 ↔ bearingsleeve_MIR1:4
- Insert:98: 608_MIR1:5 ↔ bearingsleeve_MIR1:5
- Mate:100: bearingsleeve_MIR1:5 ↔ Spur Gears4_MIR1:1
- Mate:101: Undercarriage_MIR1:1 ↔ Spur Gears4_MIR1:1
- Insert:99: Shaft LS 2.5 in:3 ↔ Shaft Collar with Set Screw_MIR1:1
- Insert:100: Pillow Bearing Block_MIR1:2 ↔ Shaft Collar with Set Screw_MIR1:1
- Insert:101: Pillow Bearing Block_MIR1:1 ↔ Shaft Collar with Set Screw_MIR1:2
- Insert:102: lower_plate_MIR1:1 ↔ 608_MIR1:6
- Insert:103: lower_plate_MIR1:1 ↔ 608_MIR1:7
- Insert:104: lower_plate_MIR1:1 ↔ 608_MIR1:8
- Insert:105: 608_MIR1:8 ↔ vroller_MIR1:1
- Mate:102: 608_MIR1:8 ↔ vroller_MIR1:1
- Mate:103: 608_MIR1:8 ↔ vroller_MIR1:1
- Mate:104: lower_plate_MIR1:1 ↔ upper_MIR1:1
- Mate:105: lower_plate_MIR1:1 ↔ upper_MIR1:1
- Mate:106: upper_MIR1:1 ↔ uppermidblock_MIR1:1
- Mate:107: upper_MIR1:1 ↔ uppermidblock_MIR1:1
- Insert:106: V5 Simple Motor_MIR1:1 ↔ motorplate_MIR1:1
- Insert:107: V5 Simple Motor_MIR1:1 ↔ motorplate_MIR1:1
- Insert:108: V5 Simple Motor_MIR1:2 ↔ motorplate_MIR1:1
- Insert:109: V5 Simple Motor_MIR1:2 ↔ motorplate_MIR1:1
- Mate:108: uppermidblock_MIR1:1 ↔ motorplate_MIR1:1
- Mate:109: Spur Gears4_MIR1:1
- Angle:9 (-90 deg): uppermidblock_MIR1:1
- Mate:110: Undercarriage_MIR1:1 ↔ encoderring_MIR1:1
- Insert:110: lower_plate_MIR1:1 ↔ Alu C 1x2x1x26_MIR:1
- Insert:111: lower_plate_MIR1:1 ↔ Alu C 1x2x1x26_MIR:2
- Insert:112: lower_plate_MIR1:1 ↔ Alu C 1x2x1x26_MIR:2
- Mate:111: Undercarriage_MIR_MIR:1 ↔ 2.75 Traction, No Insert_MIR_MIR:1
- Insert:113: Undercarriage_MIR_MIR:1 ↔ Pillow Bearing Block_MIR_MIR:1
- Insert:114: Undercarriage_MIR_MIR:1 ↔ Pillow Bearing Block_MIR_MIR:1
- Insert:115: Undercarriage_MIR_MIR:1 ↔ Pillow Bearing Block_MIR_MIR:2
- Insert:116: Undercarriage_MIR_MIR:1 ↔ Pillow Bearing Block_MIR_MIR:2
- Mate:112: Bevel Gears1_MIR2_MIR:1 ↔ Pillow Bearing Block_MIR_MIR:2
- Insert:117: Undercarriage_MIR_MIR:1 ↔ SScrew Star Smooth .750:13
- Insert:118: Undercarriage_MIR_MIR:1 ↔ SScrew Star Smooth .750:14
- Insert:119: Undercarriage_MIR_MIR:1 ↔ SScrew Star Smooth .750:15
- Insert:120: Undercarriage_MIR_MIR:1 ↔ SScrew Star Smooth .750:16
- Mate:113: Bevel Gears1_MIR2_MIR:1 ↔ Bevel Gears1_MIR1_MIR_MIR:1
- Mate:114: 2.75 Traction, No Insert_MIR_MIR:1 ↔ Bevel Gears1_MIR1_MIR_MIR:1
- Insert:121: Pillow Bearing Block_MIR_MIR:1 ↔ Nut Nylock_MIR_MIR:1
- Insert:122: Pillow Bearing Block_MIR_MIR:2 ↔ Nut Nylock_MIR_MIR:2
- Insert:123: Pillow Bearing Block_MIR_MIR:1 ↔ Nut Nylock_MIR_MIR:3
- Insert:124: Pillow Bearing Block_MIR_MIR:2 ↔ Nut Nylock_MIR_MIR:4
- Flush:12: Undercarriage_MIR_MIR:1 ↔ 608_MIR_MIR:1
- Insert:125: Undercarriage_MIR_MIR:1 ↔ 608_MIR_MIR:1
- Insert:126: Undercarriage_MIR_MIR:1 ↔ 608_MIR_MIR:2
- Insert:127: 608_MIR_MIR:2 ↔ bearingsleeve_MIR_MIR:1
- Flush:13: Undercarriage_MIR_MIR:1 ↔ lower_plate_MIR_MIR:1
- Flush:14 (3 mm): Undercarriage_MIR_MIR:1 ↔ lower_plate_MIR_MIR:1
- Mate:115: bearingsleeve_MIR_MIR:1 ↔ Spur Gears1_MIR_MIR:1
- Mate:116: Undercarriage_MIR_MIR:1 ↔ Spur Gears1_MIR_MIR:1
- Mate:117 (1.5875 mm): bearingsleeve_MIR_MIR:1 ↔ Spur Gears1_MIR_MIR:1
- Insert:128: Undercarriage_MIR_MIR:1 ↔ 608_MIR_MIR:3
- Insert:129: 608_MIR_MIR:3 ↔ bearingsleeve_MIR_MIR:2
- Mate:118 (1.5875 mm): Spur Gears1_MIR_MIR:1 ↔ bearingsleeve_MIR_MIR:2
- Insert:130: 608_MIR_MIR:1 ↔ bearingsleeve_MIR_MIR:3
- Mate:119: bearingsleeve_MIR_MIR:3 ↔ Spur Gears2_MIR_MIR:1
- Mate:120 (1.5875 mm): Spur Gears1_MIR_MIR:1 ↔ Spur Gears2_MIR_MIR:1
- Mate:121: Undercarriage_MIR_MIR:1 ↔ Spur Gears2_MIR_MIR:1
- Mate:122 (1.5875 mm): Spur Gears1_MIR_MIR:1 ↔ Spur Gears2_MIR_MIR:1
- Mate:123: Undercarriage_MIR_MIR:1 ↔ Spur Gears3_MIR_MIR:1
- Mate:124: Spur Gears2_MIR_MIR:1 ↔ Spur Gears3_MIR_MIR:1
- Insert:131: Spur Gears2_MIR_MIR:1 ↔ 608_MIR_MIR:4
- Insert:132: Spur Gears3_MIR_MIR:1 ↔ 608_MIR_MIR:5
- Insert:133: 608_MIR_MIR:4 ↔ bearingsleeve_MIR_MIR:4
- Insert:134: 608_MIR_MIR:5 ↔ bearingsleeve_MIR_MIR:5
- Mate:125: Undercarriage_MIR_MIR:1 ↔ Spur Gears4_MIR_MIR:1
- Mate:126: bearingsleeve_MIR_MIR:5 ↔ Spur Gears4_MIR_MIR:1
- Insert:135: Pillow Bearing Block_MIR_MIR:2 ↔ Shaft Collar with Set Screw_MIR_MIR:1
- Insert:136: Shaft LS 2.5 in:4 ↔ Shaft Collar with Set Screw_MIR_MIR:1
- Insert:137: Pillow Bearing Block_MIR_MIR:1 ↔ Shaft Collar with Set Screw_MIR_MIR:2
- Insert:138: lower_plate_MIR_MIR:1 ↔ 608_MIR_MIR:6
- Insert:139: lower_plate_MIR_MIR:1 ↔ 608_MIR_MIR:7
- Insert:140: lower_plate_MIR_MIR:1 ↔ 608_MIR_MIR:8
- Flush:15: 608_MIR_MIR:8 ↔ vroller_MIR_MIR:1
- Flush:16: 608_MIR_MIR:8 ↔ vroller_MIR_MIR:1
- Insert:141: 608_MIR_MIR:8 ↔ vroller_MIR_MIR:1
- Flush:17: lower_plate_MIR_MIR:1 ↔ upper_MIR_MIR:1
- Flush:18: lower_plate_MIR_MIR:1 ↔ upper_MIR_MIR:1
- Flush:19: upper_MIR_MIR:1 ↔ uppermidblock_MIR_MIR:1
- Flush:20: upper_MIR_MIR:1 ↔ uppermidblock_MIR_MIR:1
- Flush:21: uppermidblock_MIR_MIR:1 ↔ motorplate_MIR_MIR:1
- Insert:142: V5 Simple Motor_MIR_MIR:2 ↔ motorplate_MIR_MIR:1
- Insert:143: V5 Simple Motor_MIR_MIR:2 ↔ motorplate_MIR_MIR:1
- Insert:144: V5 Simple Motor_MIR_MIR:1 ↔ motorplate_MIR_MIR:1
- Insert:145: V5 Simple Motor_MIR_MIR:1 ↔ motorplate_MIR_MIR:1
- Flush:22: Undercarriage_MIR_MIR:1 ↔ encoderring_MIR_MIR:1
- Mate:127: Spur Gears4_MIR_MIR:1
- Angle:10 (0 deg): Bevel Gears1_MIR2_MIR:1 ↔ Bevel Gears1_MIR1_MIR_MIR:1
- Angle:11 (180 deg): Bevel Gears1_MIR2_MIR:1
- Angle:12 (90 deg): uppermidblock_MIR_MIR:1
- Rigid:3 [WeldJoint]: 2.75 Traction, No Insert_MIR1:1 ↔ Bevel Gears1_MIR3:1
- Rigid:4 [WeldJoint]: 2.75 Traction, No Insert_MIR_MIR:1 ↔ Bevel Gears1_MIR2_MIR:1
